# Autodesk Inventor assembly: montagemEstruturaCameraCME
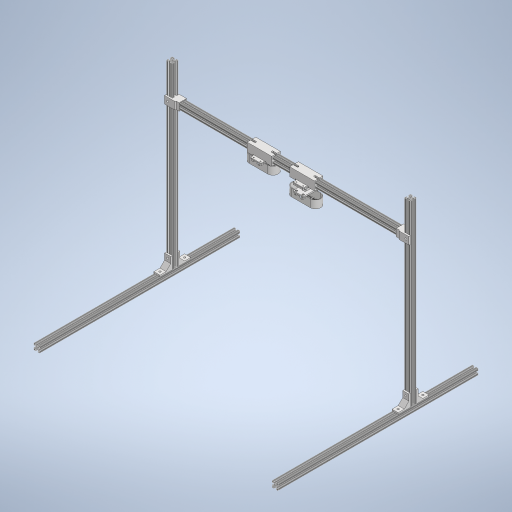
[picture p0: Inventor's stored thumbnail of the model, 512x512]
Saved by Autodesk Inventor 2023 (Build 270158000, 158)
## iProperties
Created: 2024-04-10
Part Number: montagemEstruturaCameraCME
Document SubType Name: Assembly
Designer: cvss2
Author: cvss2
## Documents named in this file (9)
- C:\Users\cvss2.CINSOFTEX\Downloads\CME - Suportes para camera\Sinaleira CME\Estrutura Camera CME\montagemEstruturaCameraCME.iam
- C:\Users\cvss2.CINSOFTEX\Downloads\CME - Suportes para camera\Sinaleira CME\Estrutura Camera CME\Perfil_Aluminio_20x20x580.ipt
- C:\Users\cvss2.CINSOFTEX\Downloads\CME - Suportes para camera\Sinaleira CME\Estrutura Camera CME\Perfil_Aluminio_20x20x650.ipt
- C:\Users\cvss2.CINSOFTEX\Downloads\CME - Suportes para camera\Sinaleira CME\Estrutura Camera CME\Perfil_Aluminio_20x20x750.ipt
- C:\Users\cvss2.CINSOFTEX\Downloads\CME - Suportes para camera\Sinaleira CME\suporteBright2k.ipt
- C:\Users\cvss2.CINSOFTEX\Downloads\CME - Suportes para camera\Sinaleira CME\Estrutura Camera CME\cantoneira.ipt
- C:\Users\cvss2.CINSOFTEX\Downloads\CME - Suportes para camera\Sinaleira CME\Estrutura Camera CME\extremidadeSlider.ipt
- C:\Users\cvss2.CINSOFTEX\Downloads\CME - Suportes para camera\Sinaleira CME\Estrutura Camera CME\cameraSlider.ipt
- C:\Users\cvss2.CINSOFTEX\Downloads\CME - Suportes para camera\Sinaleira CME\Estrutura Camera CME\encaixeDuplo.ipt
## Components (17 placed, 8 different names)
1. Perfil_Aluminio_20x20x580:1 — Mate:1, Mate:2, Flush:1, Mate:3, Flush:2, Mate:4, Flush:3, Flush:6, Flush:7, Mate:11, Mate:12, Flush:9
2. Perfil_Aluminio_20x20x580:2 — Mate:3, Flush:2, Mate:5, Flush:5, Flush:6, Mate:6, Mate:7, Mate:14, Flush:10, Mate:16, Flush:11
3. Perfil_Aluminio_20x20x650:1 — Mate:4, Flush:3, Flush:4, Mate:10, Flush:8, Mate:13
4. Perfil_Aluminio_20x20x650:2 — Flush:4, Mate:5, Flush:5, Mate:6, Mate:15, Mate:17
5. Perfil_Aluminio_20x20x750:1 — Flush:7, Mate:7, Mate:18, Mate:19, Mate:20, Mate:21, Mate:22, Mate:23, Mate:24, Mate:25, Mate:31, Mate:32
6. cantoneira:1 — Mate:10, Flush:8, Mate:11
7. cantoneira:2 — Mate:12, Mate:13, Flush:9
8. cantoneira:3 — Mate:14, Flush:10, Mate:15
9. cantoneira:4 — Mate:16, Mate:17, Flush:11
10. extremidadeSlider:1 — Mate:18, Mate:19, Mate:20
11. extremidadeSlider:2 — Mate:21, Mate:22, Mate:23
12. cameraSlider:1 — Mate:24, Mate:25, Mate:26, Mate:27, Mate:28
13. suporteBright2k:1 — Mate:26, Mate:27, Mate:28
14. cameraSlider:2 — Mate:31, Mate:32, Mate:33, Mate:34, Mate:35
15. encaixeDuplo:1 — Mate:29, Mate:30, Mate:33, Mate:34, Mate:35
16. encaixeDuplo:2 — Mate:29, Mate:30, Mate:36, Mate:37, Mate:38
17. suporteBright2k:2 — Mate:36, Mate:37, Mate:38
## Relationships (47: Mate 36, Flush 11)
- Mate:1: Perfil_Aluminio_20x20x580:1
- Mate:2: Perfil_Aluminio_20x20x580:1
- Flush:1: Perfil_Aluminio_20x20x580:1
- Mate:3 (754 mm): Perfil_Aluminio_20x20x580:1 ↔ Perfil_Aluminio_20x20x580:2
- Flush:2: Perfil_Aluminio_20x20x580:1 ↔ Perfil_Aluminio_20x20x580:2
- Mate:4: Perfil_Aluminio_20x20x580:1 ↔ Perfil_Aluminio_20x20x650:1
- Flush:3: Perfil_Aluminio_20x20x580:1 ↔ Perfil_Aluminio_20x20x650:1
- Flush:4: Perfil_Aluminio_20x20x650:1 ↔ Perfil_Aluminio_20x20x650:2
- Mate:5: Perfil_Aluminio_20x20x580:2 ↔ Perfil_Aluminio_20x20x650:2
- Flush:5: Perfil_Aluminio_20x20x580:2 ↔ Perfil_Aluminio_20x20x650:2
- Flush:6: Perfil_Aluminio_20x20x580:1 ↔ Perfil_Aluminio_20x20x580:2
- Mate:6 (-220 mm): Perfil_Aluminio_20x20x580:2 ↔ Perfil_Aluminio_20x20x650:2
- Flush:7: Perfil_Aluminio_20x20x580:1 ↔ Perfil_Aluminio_20x20x750:1
- Mate:7 (2 mm): Perfil_Aluminio_20x20x580:2 ↔ Perfil_Aluminio_20x20x750:1
- Mate:10: Perfil_Aluminio_20x20x650:1 ↔ cantoneira:1
- Flush:8: Perfil_Aluminio_20x20x650:1 ↔ cantoneira:1
- Mate:11: Perfil_Aluminio_20x20x580:1 ↔ cantoneira:1
- Mate:12: Perfil_Aluminio_20x20x580:1 ↔ cantoneira:2
- Mate:13: Perfil_Aluminio_20x20x650:1 ↔ cantoneira:2
- Flush:9: Perfil_Aluminio_20x20x580:1 ↔ cantoneira:2
- Mate:14: Perfil_Aluminio_20x20x580:2 ↔ cantoneira:3
- Flush:10: Perfil_Aluminio_20x20x580:2 ↔ cantoneira:3
- Mate:15: Perfil_Aluminio_20x20x650:2 ↔ cantoneira:3
- Mate:16: Perfil_Aluminio_20x20x580:2 ↔ cantoneira:4
- Mate:17: Perfil_Aluminio_20x20x650:2 ↔ cantoneira:4
- Flush:11: Perfil_Aluminio_20x20x580:2 ↔ cantoneira:4
- Mate:18: Perfil_Aluminio_20x20x750:1 ↔ extremidadeSlider:1
- Mate:19: Perfil_Aluminio_20x20x750:1 ↔ extremidadeSlider:1
- Mate:20: Perfil_Aluminio_20x20x750:1 ↔ extremidadeSlider:1
- Mate:21: Perfil_Aluminio_20x20x750:1 ↔ extremidadeSlider:2
- Mate:22: Perfil_Aluminio_20x20x750:1 ↔ extremidadeSlider:2
- Mate:23: Perfil_Aluminio_20x20x750:1 ↔ extremidadeSlider:2
- Mate:24: Perfil_Aluminio_20x20x750:1 ↔ cameraSlider:1
- Mate:25: Perfil_Aluminio_20x20x750:1 ↔ cameraSlider:1
- Mate:26: cameraSlider:1 ↔ suporteBright2k:1
- Mate:27: cameraSlider:1 ↔ suporteBright2k:1
- Mate:28: cameraSlider:1 ↔ suporteBright2k:1
- Mate:29: encaixeDuplo:1 ↔ encaixeDuplo:2
- Mate:30 (0.1 mm): encaixeDuplo:1 ↔ encaixeDuplo:2
- Mate:31: Perfil_Aluminio_20x20x750:1 ↔ cameraSlider:2
- Mate:32: Perfil_Aluminio_20x20x750:1 ↔ cameraSlider:2
- Mate:33: cameraSlider:2 ↔ encaixeDuplo:1
- Mate:34: cameraSlider:2 ↔ encaixeDuplo:1
- Mate:35: cameraSlider:2 ↔ encaixeDuplo:1
- Mate:36: encaixeDuplo:2 ↔ suporteBright2k:2
- Mate:37: encaixeDuplo:2 ↔ suporteBright2k:2
- Mate:38: encaixeDuplo:2 ↔ suporteBright2k:2
